# Autodesk Inventor assembly: splitter_all
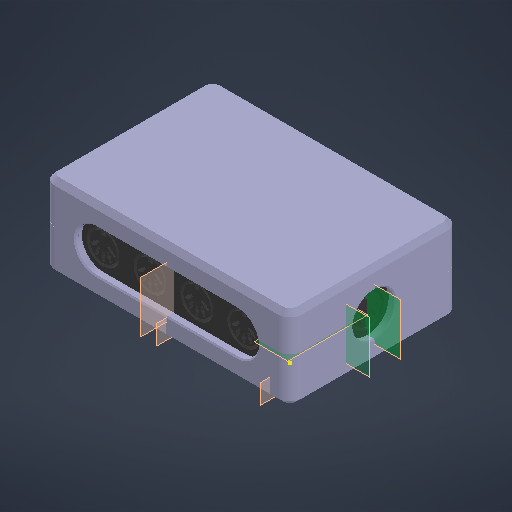
[picture p0: Inventor's stored thumbnail of the model, 512x512]
Saved by Autodesk Inventor 2025.2 (Build 292293000, 293)
## iProperties
Created: 2025-10-04
Part Number: splitter_all
Document SubType Name: Assembly
Designer: micyg
Author: micyg
## Documents named in this file (5)
- D:\Projects\AnotherMidiSplitterV2\Mechanical\splitter_all.iam
- D:\Projects\AnotherMidiSplitterV2\Mechanical\case2.ipt
- D:\Projects\AnotherMidiSplitterV2\Mechanical\mounting.ipt
- D:\Projects\AnotherMidiSplitterV2\Mechanical\Boards\AnotherMidiSplitterV2\AnotherMidiSplitterV2.iam
- D:\Projects\AnotherMidiSplitterV2\Mechanical\case1.ipt
## Components (7 placed, 4 different names)
1. case1:1 — Mate:12, Mate:13, Mate:14
2. case2:1 — Mate:1, Mate:2, Mate:3, Mate:4, Mate:5, Mate:6, Mate:7, Mate:8, Mate:14
3. mounting:1 — Mate:1, Mate:2, Mate:10
4. AnotherMidiSplitterV2:1 [sub-assembly] — Mate:9, Mate:10, Mate:11, Mate:12, Mate:13
5. mounting:2 — Mate:5, Mate:6
6. mounting:3 — Mate:4, Mate:8, Mate:9
7. mounting:4 — Mate:3, Mate:7, Mate:11
## Relationships (14: Mate 14)
- Mate:1: case2:1 ↔ mounting:1
- Mate:2: case2:1 ↔ mounting:1
- Mate:3: case2:1 ↔ mounting:4
- Mate:4: case2:1 ↔ mounting:3
- Mate:5: case2:1 ↔ mounting:2
- Mate:6: case2:1 ↔ mounting:2
- Mate:7: case2:1 ↔ mounting:4
- Mate:8: case2:1 ↔ mounting:3
- Mate:9: AnotherMidiSplitterV2:1 ↔ mounting:3
- Mate:10: mounting:1 ↔ AnotherMidiSplitterV2:1
- Mate:11: AnotherMidiSplitterV2:1 ↔ mounting:4
- Mate:12: case1:1 ↔ AnotherMidiSplitterV2:1
- Mate:13: case1:1 ↔ AnotherMidiSplitterV2:1
- Mate:14: case1:1 ↔ case2:1
